# Autodesk Inventor assembly: X_CarriageL_V2_0_Short
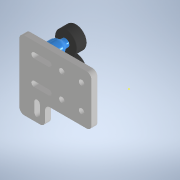
[picture p0: Inventor's stored thumbnail of the model, 180x180]
Saved by Autodesk Inventor 2021 (Build 250183000, 183)
## iProperties
Created: 2021-06-13
Part Number: X_CarriageL_V2_0_Short
Document SubType Name: Assembly
Designer: Jorian Brusind
Author: Jorian Brusind
## Documents named in this file (4)
- C:\Users\Jorian Brusind\Documents\GitHub\PersonalProjects\HyperRail\Inventor Files\X_CarriageL_V2_0_Short.iam
- C:\Users\Jorian Brusind\Documents\GitHub\PersonalProjects\HyperRail\Inventor Files\11mm_BearingWheel.ipt
- C:\Users\Jorian Brusind\Documents\GitHub\PersonalProjects\HyperRail\Inventor Files\4mm_Roller_Spacer_simple.ipt
- C:\Users\Jorian Brusind\Documents\GitHub\PersonalProjects\HyperRail\Inventor Files\X_Carriage_Plate_Short.ipt
## Components (4 placed, 3 different names)
1. 11mm_BearingWheel:2 — Flush:1, Mate:3, Mate:4
2. 11mm_BearingWheel:3 — Flush:1, Mate:5
3. X_Carriage_Plate_Short:1 — Mate:6, Mate:7, Angle:1
4. 4mm_Roller_Spacer_simple:1 — Mate:3, Mate:4, Mate:5, Mate:6, Mate:7, Angle:1
## Relationships (7: Mate 5, Flush 1, Angle 1)
- Flush:1: 11mm_BearingWheel:2 ↔ 11mm_BearingWheel:3
- Mate:3: 11mm_BearingWheel:2 ↔ 4mm_Roller_Spacer_simple:1
- Mate:4: 11mm_BearingWheel:2 ↔ 4mm_Roller_Spacer_simple:1
- Mate:5: 11mm_BearingWheel:3 ↔ 4mm_Roller_Spacer_simple:1
- Mate:6: X_Carriage_Plate_Short:1 ↔ 4mm_Roller_Spacer_simple:1
- Mate:7 (-12.5 mm): X_Carriage_Plate_Short:1 ↔ 4mm_Roller_Spacer_simple:1
- Angle:1 (0 deg): X_Carriage_Plate_Short:1 ↔ 4mm_Roller_Spacer_simple:1
